# Autodesk Inventor assembly: señales_Assembly_x10
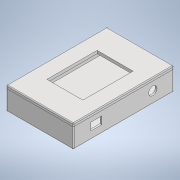
[picture p0: Inventor's stored thumbnail of the model, 180x180]
Saved by Autodesk Inventor 2022 (Build 260153000, 153)
## iProperties
Created: 2023-07-04
Part Number: señales_Assembly_x10
Document SubType Name: Assembly
Designer: Asus
Author: Asus
## Documents named in this file (3)
- C:\Users\Asus\Documents\señales_Assembly_x10.iam
- C:\Users\Asus\Documents\señales_carcasa_x10.ipt
- C:\Users\Asus\Documents\señales_tapa_x10.ipt
## Components (2 placed, 2 different names)
1. señales_carcasa_x10:1 — Mate:1, Flush:1, Flush:2
2. señales_tapa_x10:1 — Mate:1, Flush:1, Flush:2
## Relationships (3: Flush 2, Mate 1)
- Mate:1: señales_carcasa_x10:1 ↔ señales_tapa_x10:1
- Flush:1: señales_carcasa_x10:1 ↔ señales_tapa_x10:1
- Flush:2: señales_carcasa_x10:1 ↔ señales_tapa_x10:1
